# Autodesk Inventor assembly: DeadWheelAssembly
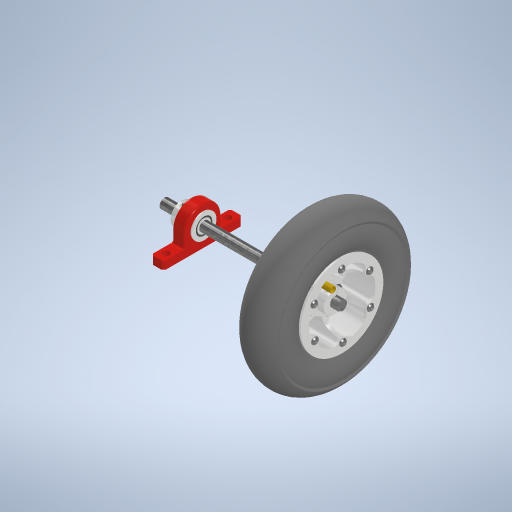
[picture p0: Inventor's stored thumbnail of the model, 512x512]
Saved by Autodesk Inventor 2023 (Build 270158000, 158)
## iProperties
Created: 2022-09-14
Part Number: DeadWheelAssembly
Document SubType Name: Assembly
Designer: PC
Author: PC
## Documents named in this file (6)
- C:\Users\PC\Documents\PersonalCAD\ARCIGVC\IGVC-Robot\DeadWheelAssembly.iam
- C:\Users\PC\Documents\PersonalCAD\ARCIGVC\IGVC-Robot\Bearing Housing.ipt
- C:\Users\PC\Documents\PersonalCAD\ARCIGVC\IGVC-Robot\half in Bearing Flanged.ipt
- C:\Users\PC\Documents\PersonalCAD\ARCIGVC\IGVC-Robot\8inPneumaticDEAD.ipt
- C:\Users\PC\Documents\PersonalCAD\ARCIGVC\IGVC-Robot\SteelDeadAxel.ipt
- C:\Users\PC\Documents\PersonalCAD\ARCIGVC\IGVC-Robot\am-2099 Collar Clamp, 0.5'' Bore, Aluminum.ipt
## Components (12 placed, 5 different names)
1. Bearing Housing:1 — Flush:2, Flush:3
2. Bearing Housing:2 — Flush:2
3. half in Bearing Flanged:1
4. half in Bearing Flanged:2
5. half in Bearing Flanged:3
6. half in Bearing Flanged:4
7. 8inPneumaticDEAD:1
8. half in Bearing Flanged:5
9. half in Bearing Flanged:6
10. SteelDeadAxel:1 — Flush:3
11. am-2099 Collar Clamp, 0.5'' Bore, Aluminum:1
12. am-2099 Collar Clamp, 0.5'' Bore, Aluminum:2
## Relationships (23: Mate 20, Flush 3)
- [Mate]: Bearing Housing:1 ↔ Bearing Housing:2
- [Mate]: Bearing Housing:2 ↔ half in Bearing Flanged:2
- [Mate]: Bearing Housing:1 ↔ half in Bearing Flanged:3
- [Mate]: Bearing Housing:2 ↔ half in Bearing Flanged:4
- [Mate]: Bearing Housing:1 ↔ half in Bearing Flanged:1
- [Mate]: Bearing Housing:1 ↔ half in Bearing Flanged:1
- [Mate]: Bearing Housing:1 ↔ half in Bearing Flanged:3
- [Mate]: Bearing Housing:2 ↔ half in Bearing Flanged:4
- [Mate]: Bearing Housing:2 ↔ half in Bearing Flanged:2
- [Mate]: 8inPneumaticDEAD:1 ↔ half in Bearing Flanged:6
- [Mate]: 8inPneumaticDEAD:1 ↔ half in Bearing Flanged:6
- [Mate]: 8inPneumaticDEAD:1 ↔ half in Bearing Flanged:5
- [Mate]: 8inPneumaticDEAD:1 ↔ half in Bearing Flanged:5
- [Mate]: half in Bearing Flanged:2 ↔ half in Bearing Flanged:6
- [Mate] (12.7 mm): half in Bearing Flanged:2 ↔ half in Bearing Flanged:6
- [Flush]: 8inPneumaticDEAD:1 ↔ SteelDeadAxel:1
- [Mate]: half in Bearing Flanged:5 ↔ SteelDeadAxel:1
- [Mate]: SteelDeadAxel:1 ↔ am-2099 Collar Clamp, 0.5'' Bore, Aluminum:1
- [Mate]: half in Bearing Flanged:5 ↔ am-2099 Collar Clamp, 0.5'' Bore, Aluminum:1
- [Mate]: SteelDeadAxel:1 ↔ am-2099 Collar Clamp, 0.5'' Bore, Aluminum:2
- [Mate]: half in Bearing Flanged:1 ↔ am-2099 Collar Clamp, 0.5'' Bore, Aluminum:2
- Flush:2: Bearing Housing:1 ↔ Bearing Housing:2
- Flush:3 (33.655 mm): Bearing Housing:1 ↔ SteelDeadAxel:1
## Named parameters: d165_d114_d66 = 0 mm
